# Autodesk Inventor assembly: gusset_roofFloor
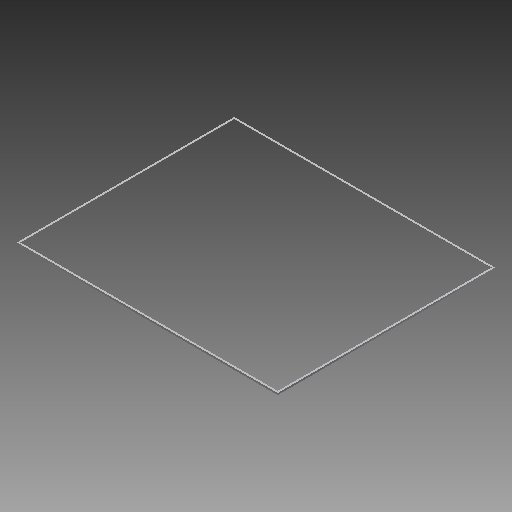
[picture p0: Inventor's stored thumbnail of the model, 512x512]
Saved by Autodesk Inventor 2019 (Build 230136000, 136)
## iProperties
Created: 2018-07-11
Part Number: gusset_roofFloor
Document SubType Name: Assembly
Designer: User
Author: User
## Documents named in this file (5)
- C:\Users\phys-simulation\Desktop\DarkRadioSimulations\3D Models\Room Model\gusset_roofFloor.iam
- C:\Users\phys-simulation\Desktop\DarkRadioSimulations\3D Models\Room Model\gusset_plate_leftRight.ipt
- C:\Users\phys-simulation\Desktop\DarkRadioSimulations\3D Models\Room Model\gusset_plate_corner.ipt
- C:\Users\phys-simulation\Desktop\DarkRadioSimulations\3D Models\Room Model\gusset_plate_frontBack.ipt
- C:\Users\phys-simulation\Desktop\DarkRadioSimulations\3D Models\Room Model\params.xlsx
## Components (8 placed, 3 different names)
1. gusset_plate_leftRight:1 — Rigid:1, Rigid:2
2. gusset_plate_corner:1 — Rigid:1
3. gusset_plate_corner:2 — Rigid:2, Rigid:3
4. gusset_plate_frontBack:1 — Rigid:3, Rigid:4
5. gusset_plate_corner:3 — Rigid:4, Rigid:5
6. gusset_plate_leftRight:2 — Rigid:5, Rigid:6
7. gusset_plate_corner:4 — Rigid:6, Rigid:7
8. gusset_plate_frontBack:2 — Rigid:7
## Relationships (7: WeldJoint 7)
- Rigid:1 [WeldJoint]: gusset_plate_leftRight:1 ↔ gusset_plate_corner:1
- Rigid:2 [WeldJoint]: gusset_plate_leftRight:1 ↔ gusset_plate_corner:2
- Rigid:3 [WeldJoint]: gusset_plate_corner:2 ↔ gusset_plate_frontBack:1
- Rigid:4 [WeldJoint]: gusset_plate_frontBack:1 ↔ gusset_plate_corner:3
- Rigid:5 [WeldJoint]: gusset_plate_corner:3 ↔ gusset_plate_leftRight:2
- Rigid:6 [WeldJoint]: gusset_plate_leftRight:2 ↔ gusset_plate_corner:4
- Rigid:7 [WeldJoint]: gusset_plate_corner:4 ↔ gusset_plate_frontBack:2
## Named parameters: wallThick = 44.45 mm, roomWidth = 3048 mm, roomDepth = 3657.6 mm, roomHeight = 2438.4 mm, doorWidth = 895.35 mm, doorHeight = 2108.2 mm, doorX = 774.7 mm, doorY = 88.9 mm, doorLip = 76.2 mm, doorThick = 57.15 mm, tubeD = 19.05 mm, tubeTurnR = 76.2 mm
